# Autodesk Inventor assembly: bashnia
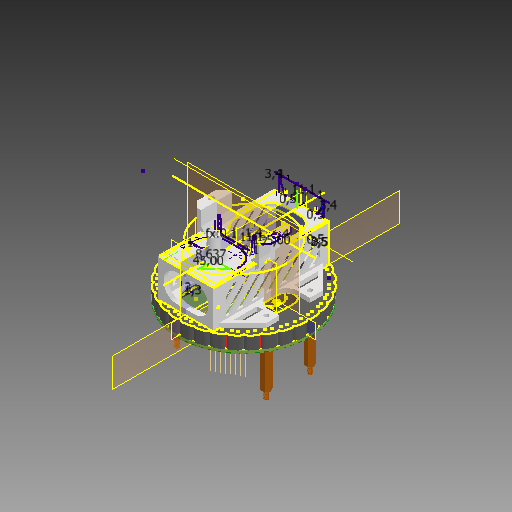
[picture p0: Inventor's stored thumbnail of the model, 512x512]
Saved by Autodesk Inventor 2020 (Build 240168000, 168)
## iProperties
Created: 2024-12-27
Part Number: bashnia
Document SubType Name: Assembly
Designer: Ivan
Author: Ivan
## Documents named in this file (5)
- C:\!projects\DASH-\3D\Dash-V1\bashnia\bashnia.iam
- C:\!projects\DASH-\3D\Dash-V1\tsop.iam
- C:\!projects\DASH-\3D\Dash-V1\step\akb_m\akb_mount1550.ipt
- C:\!projects\DASH-\3D\Dash-V1\step\m3_bolt\Spacer Bolts_m3_bn_L25.ipt
- C:\!projects\DASH-\3D\Dash-V1\step\lpls\DS1021_black_1x04p_100mil_Type43_rev1.0.ipt
## Components (8 placed, 4 different names)
1. tsop:1 [sub-assembly] — Совмещение:1, Совмещение:2, Вставка:1, Заподлицо:1, Вставка:2, Вставка:3, Вставка:4, Вставка:5, Совмещение:4, Угол:4
2. akb_mount1550:1 — Угол:2, Вставка:1, Заподлицо:1
3. Spacer Bolts_m3_bn_L30:1 — Вставка:2
4. Spacer Bolts_m3_bn_L30:2 — Вставка:3
5. Spacer Bolts_m3_bn_L30:3 — Вставка:4
6. Spacer Bolts_m3_bn_L30:4 — Вставка:5, Угол:4
7. DS1021_black_1x04p_100mil_Type43_rev1.0:1 — Совмещение:3, Заподлицо:2, Заподлицо:3, Угол:3
8. DS1021_black_1x04p_100mil_Type43_rev1.0:2 — Совмещение:3, Заподлицо:2, Заподлицо:3, Совмещение:4
## Relationships (15: Insert 5, Mate 4, Angle 3, Flush 3)
- Совмещение:1 [Mate]: tsop:1
- Совмещение:2 [Mate]: tsop:1
- Угол:2 [Angle] (0 deg): akb_mount1550:1
- Вставка:1 [Insert]: tsop:1 ↔ akb_mount1550:1
- Заподлицо:1 [Flush]: tsop:1 ↔ akb_mount1550:1
- Вставка:2 [Insert]: tsop:1 ↔ Spacer Bolts_m3_bn_L30:1
- Вставка:3 [Insert]: tsop:1 ↔ Spacer Bolts_m3_bn_L30:2
- Вставка:4 [Insert]: tsop:1 ↔ Spacer Bolts_m3_bn_L30:3
- Вставка:5 [Insert]: tsop:1 ↔ Spacer Bolts_m3_bn_L30:4
- Совмещение:3 [Mate]: DS1021_black_1x04p_100mil_Type43_rev1.0:1 ↔ DS1021_black_1x04p_100mil_Type43_rev1.0:2
- Заподлицо:2 [Flush]: DS1021_black_1x04p_100mil_Type43_rev1.0:1 ↔ DS1021_black_1x04p_100mil_Type43_rev1.0:2
- Заподлицо:3 [Flush]: DS1021_black_1x04p_100mil_Type43_rev1.0:1 ↔ DS1021_black_1x04p_100mil_Type43_rev1.0:2
- Совмещение:4 [Mate]: tsop:1 ↔ DS1021_black_1x04p_100mil_Type43_rev1.0:2
- Угол:3 [Angle] (60 deg): DS1021_black_1x04p_100mil_Type43_rev1.0:1
- Угол:4 [Angle] (0 deg): tsop:1 ↔ Spacer Bolts_m3_bn_L30:4
